# Autodesk Inventor assembly: KND-2600 DrainSystemBottom 01
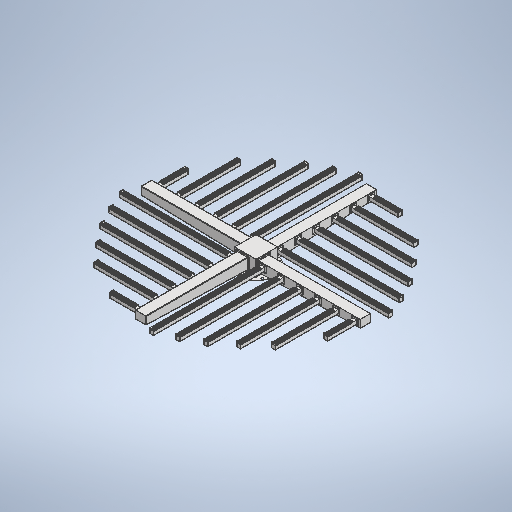
[picture p0: Inventor's stored thumbnail of the model, 512x512]
Saved by Autodesk Inventor 2026.2 (Build 302298000, 298)
## iProperties
Created: 2026-05-12
Part Number: KND-2600 DrainSystemBottom 01
Document SubType Name: Assembly
Designer: admin
Author: admin
## Documents named in this file (6)
- C:\Users\admin\Documents\Inventor\KND-DistribSystem\DRS_D1200\KND-2600 DrainSystemBottom 01.iam
- C:\Users\admin\Documents\Inventor\KND-DistribSystem\DRS_D1200\KND-9651 DrSysB MAIN FLANGE 01.ipt
- C:\Users\admin\Documents\Inventor\KND-DistribSystem\DRS_D1200\KND-1401 DrSysB DIMentions 01.ipt
- C:\Users\admin\Documents\Inventor\KND-DistribSystem\DRS_D1200\KND-1652 DrSysB Central tube wall 01.ipt
- C:\Users\admin\Documents\Inventor\KND-DistribSystem\DRS_D1200\KND-1665 DrSysB CUP 1 01.ipt
- C:\Users\admin\Documents\Inventor\KND-DistribSystem\DRS_D1200\KND-2610 Main way 01.iam
## Components (10 placed, 6 different names)
1. PRS 9651 DrSysB MAIN  FLANGE_D1200:1 — Flush:8, Flush:7, Mate:3
2. PRS 1401 DrSysB DIMentions_D1200:1
3. PRS 1652 DrSysB Central tube wall_D1200:1 — Flush:8, Flush:7, Mate:10, Rigid:22, Mate:6, Mate:7, Mate:8, Mate:9, Mate:10, Mate:11
4. PRS 1652 DrSysB Central tube wall_D1200:2 — Mate:3, Rigid:22, Mate:12, Mate:13, Mate:14, Mate:15, Mate:16, Mate:17
5. PRS 1665 DrSysB CUP 1_D1200:1 — Mate:10
6. KND-1401 DrSysB DIMentions 01:2
7. KND-2610 Main way 01:1 [sub-assembly] — Mate:6, Mate:7, Mate:8
8. KND-2610 Main way 01:2 [sub-assembly] — Mate:9, Mate:10, Mate:11
9. KND-2610 Main way 01:3 [sub-assembly] — Mate:12, Mate:13, Mate:14
10. KND-2610 Main way 01:4 [sub-assembly] — Mate:15, Mate:16, Mate:17
## Relationships (17: Mate 14, Flush 2, WeldJoint 1)
- Flush:8: PRS 9651 DrSysB MAIN  FLANGE_D1200:1 ↔ PRS 1652 DrSysB Central tube wall_D1200:1
- Flush:7: PRS 9651 DrSysB MAIN  FLANGE_D1200:1 ↔ PRS 1652 DrSysB Central tube wall_D1200:1
- Mate:10: PRS 1652 DrSysB Central tube wall_D1200:1 ↔ PRS 1665 DrSysB CUP 1_D1200:1
- Mate:3: PRS 9651 DrSysB MAIN  FLANGE_D1200:1 ↔ PRS 1652 DrSysB Central tube wall_D1200:2
- Rigid:22 [WeldJoint]: PRS 1652 DrSysB Central tube wall_D1200:1 ↔ PRS 1652 DrSysB Central tube wall_D1200:2
- Mate:6: PRS 1652 DrSysB Central tube wall_D1200:1 ↔ KND-2610 Main way 01:1
- Mate:7 (0.3 mm): PRS 1652 DrSysB Central tube wall_D1200:1 ↔ KND-2610 Main way 01:1
- Mate:8 (0.25 mm): PRS 1652 DrSysB Central tube wall_D1200:1 ↔ KND-2610 Main way 01:1
- Mate:9: PRS 1652 DrSysB Central tube wall_D1200:1 ↔ KND-2610 Main way 01:2
- Mate:10 (0.2 mm): PRS 1652 DrSysB Central tube wall_D1200:1 ↔ KND-2610 Main way 01:2
- Mate:11 (0.25 mm): PRS 1652 DrSysB Central tube wall_D1200:1 ↔ KND-2610 Main way 01:2
- Mate:12: PRS 1652 DrSysB Central tube wall_D1200:2 ↔ KND-2610 Main way 01:3
- Mate:13 (0.2 mm): PRS 1652 DrSysB Central tube wall_D1200:2 ↔ KND-2610 Main way 01:3
- Mate:14 (0.3 mm): PRS 1652 DrSysB Central tube wall_D1200:2 ↔ KND-2610 Main way 01:3
- Mate:15: PRS 1652 DrSysB Central tube wall_D1200:2 ↔ KND-2610 Main way 01:4
- Mate:16 (0.2 mm): PRS 1652 DrSysB Central tube wall_D1200:2 ↔ KND-2610 Main way 01:4
- Mate:17 (0.3 mm): PRS 1652 DrSysB Central tube wall_D1200:2 ↔ KND-2610 Main way 01:4
